# Autodesk Inventor assembly: Lander
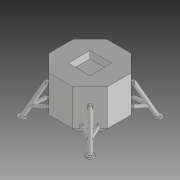
[picture p0: Inventor's stored thumbnail of the model, 180x180]
Saved by Autodesk Inventor 2020 (Build 240168000, 168)
## iProperties
Created: 2021-03-26
Part Number: Lander
Document SubType Name: Assembly
Designer: DDeGo
Author: DDeGo
## Documents named in this file (4)
- C:\Users\DDeGo\Documents\Drew\Projects\VariLev\cad\Lander\Lander.iam
- C:\Users\DDeGo\Documents\Drew\Projects\VariLev\cad\Lander\Body.ipt
- C:\Users\DDeGo\Documents\Drew\Projects\VariLev\cad\Lander\Leg.ipt
- C:\Users\DDeGo\Documents\Drew\Projects\VariLev\cad\Lander\Magnet.ipt
## Components (6 placed, 3 different names)
1. Body:1 — Mate:1, Mate:2, Mate:3, Mate:4, Mate:5, Mate:6, Mate:7, Mate:8, Mate:9, Mate:10, Mate:11, Mate:12, Mate:13, Mate:14
2. Leg:1 — Mate:3, Mate:4, Mate:5
3. Leg:2 — Mate:6, Mate:7, Mate:8
4. Leg:3 — Mate:9, Mate:10, Mate:11
5. Leg:4 — Mate:12, Mate:13, Mate:14
6. Magnet:1 — Mate:1, Mate:2
## Relationships (14: Mate 14)
- Mate:1: Body:1 ↔ Magnet:1
- Mate:2: Body:1 ↔ Magnet:1
- Mate:3: Body:1 ↔ Leg:1
- Mate:4: Body:1 ↔ Leg:1
- Mate:5: Body:1 ↔ Leg:1
- Mate:6: Body:1 ↔ Leg:2
- Mate:7: Body:1 ↔ Leg:2
- Mate:8: Body:1 ↔ Leg:2
- Mate:9: Body:1 ↔ Leg:3
- Mate:10: Body:1 ↔ Leg:3
- Mate:11: Body:1 ↔ Leg:3
- Mate:12: Body:1 ↔ Leg:4
- Mate:13: Body:1 ↔ Leg:4
- Mate:14: Body:1 ↔ Leg:4
